# Autodesk Inventor assembly: routerplatebuying
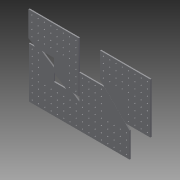
[picture p0: Inventor's stored thumbnail of the model, 180x180]
Saved by Autodesk Inventor 2014 (Build 180170000, 170)
## iProperties
Created: 2014-10-17
Part Number: routerplatebuying
Document SubType Name: Assembly
Designer: Matthew
Author: Matthew
## Documents named in this file (3)
- C:\Users\Matthew\Documents\GitHub\CNC Mill\8020\routerplatebuying.iam
- C:\Users\Matthew\Documents\GitHub\CNC Mill\8020\2020-2040_mounting_plate.ipt
- C:\Users\Matthew\Documents\GitHub\CNC Mill\8020\2040-2040_mounting_plate.ipt
## Components (4 placed, 2 different names)
1. 2020-2040_mounting_plate:1 — Mate:1, Mate:2, Flush:1, Flush:4
2. 2040-2040_mounting_plate:1 — Mate:3, Flush:2, Flush:5, Mate:4
3. 2020-2040_mounting_plate:2 — Mate:1, Mate:2, Flush:1, Flush:2, Mate:4
4. 2040-2040_mounting_plate:2 — Mate:3, Flush:4, Flush:5
## Relationships (8: Mate 4, Flush 4)
- Mate:1: 2020-2040_mounting_plate:1 ↔ 2020-2040_mounting_plate:2
- Mate:2: 2020-2040_mounting_plate:1 ↔ 2020-2040_mounting_plate:2
- Flush:1: 2020-2040_mounting_plate:1 ↔ 2020-2040_mounting_plate:2
- Mate:3: 2040-2040_mounting_plate:1 ↔ 2040-2040_mounting_plate:2
- Flush:2: 2040-2040_mounting_plate:1 ↔ 2020-2040_mounting_plate:2
- Flush:4: 2020-2040_mounting_plate:1 ↔ 2040-2040_mounting_plate:2
- Flush:5: 2040-2040_mounting_plate:1 ↔ 2040-2040_mounting_plate:2
- Mate:4: 2040-2040_mounting_plate:1 ↔ 2020-2040_mounting_plate:2
